# Autodesk Inventor assembly: 팔각형 OV-PAM 5패턴
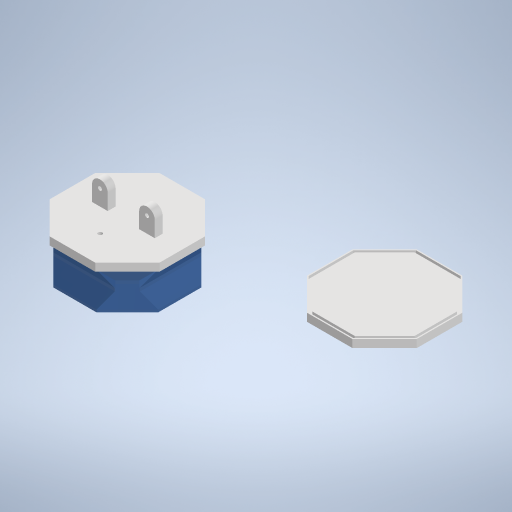
[picture p0: Inventor's stored thumbnail of the model, 512x512]
Saved by Autodesk Inventor 2024 (Build 280153000, 153)
## iProperties
Created: 2023-06-16
Part Number: 팔각형 OV-PAM 5패턴
Document SubType Name: Assembly
Designer: jsw
Author: jsw
## Documents named in this file (4)
- C:\승원\co-op\OV-PAM\OV-PAM_modeling\OV-PAM_5_patterns.iam
- C:\승원\co-op\OV-PAM\OV-PAM_modeling\OV-PAM_5_patterns_1f.ipt
- C:\승원\co-op\OV-PAM\OV-PAM_modeling\OV-PAM_top.ipt
- C:\승원\co-op\OV-PAM\OV-PAM_modeling\OV-PAM_bottom.ipt
## Components (3 placed, 3 different names)
1. OV-PAM_5_patterns_1f:1 — 메이트:1, 메이트:2, 메이트:3
2. OV-PAM_top:1 — 메이트:1, 메이트:2, 메이트:3
3. OV-PAM_bottom:1
## Relationships (3: Mate 3)
- 메이트:1 [Mate]: OV-PAM_5_patterns_1f:1 ↔ OV-PAM_top:1
- 메이트:2 [Mate]: OV-PAM_5_patterns_1f:1 ↔ OV-PAM_top:1
- 메이트:3 [Mate]: OV-PAM_5_patterns_1f:1 ↔ OV-PAM_top:1
